# Autodesk Inventor assembly: Assembly
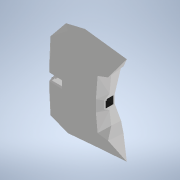
[picture p0: Inventor's stored thumbnail of the model, 180x180]
Saved by Autodesk Inventor 2020 (Build 240168000, 168)
## iProperties
Created: 2020-04-24
Part Number: Assembly
Document SubType Name: Assembly
Designer: atmat
Author: atmat
## Documents named in this file (3)
- D:\1.Projects\1.Roboty\5.Micromouse\Czesci\Assembly.iam
- D:\1.Projects\2.Konsola\1.Joystick v2\Czesci\Obudowa_v1_SHELL_1.ipt
- D:\1.Projects\2.Konsola\1.Joystick v2\Czesci\Obudowa_v1_srodek_2d.ipt
## Components (2 placed, 2 different names)
1. Obudowa_v1_SHELL_1:1 — Flush:1, Flush:2, Flush:3
2. Obudowa_v1_srodek_2d:1 — Flush:4, Flush:5, Flush:6
## Relationships (6: Flush 6)
- Flush:1: Obudowa_v1_SHELL_1:1
- Flush:2: Obudowa_v1_SHELL_1:1
- Flush:3: Obudowa_v1_SHELL_1:1
- Flush:4: Obudowa_v1_srodek_2d:1
- Flush:5: Obudowa_v1_srodek_2d:1
- Flush:6: Obudowa_v1_srodek_2d:1
